# Autodesk Inventor assembly: BackMountAssembly_SimplfiedVersion_MIR
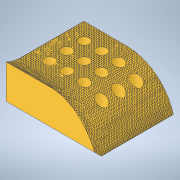
[picture p0: Inventor's stored thumbnail of the model, 180x180]
Saved by Autodesk Inventor 2021 (Build 250183000, 183)
## iProperties
Created: 2019-05-05
Part Number: BackMountAssembly_SimplfiedVersion_MIR
Document SubType Name: Assembly
Designer: CASE-SMALL2
Author: lgnds
## Documents named in this file (2)
- C:\Users\Viktor\Google Drive\Chalmers\Fortsatt arbete WR\Design files\FRS - Front Rail System_V2\FästenFörRam\BackMountAssembly_SimplfiedVersion_MIR.iam
- C:\Users\Viktor\Google Drive\Chalmers\Fortsatt arbete WR\Design files\FRS - Front Rail System_V2\FästenFörRam\BakV4_SimplifiedVersionV2_MIR.ipt
## Components (1 placed, 1 different names)
1. BakV4_SimplifiedVersionV2_MIR:1 — Flush:2, Flush:1, Mate:1
## Relationships (3: Mate 2, Flush 1)
- Flush:2 [Mate] (-45 mm): BakV4_SimplifiedVersionV2_MIR:1
- Flush:1 (58 mm): BakV4_SimplifiedVersionV2_MIR:1
- Mate:1 (183 mm): BakV4_SimplifiedVersionV2_MIR:1
